# Autodesk Inventor assembly: ShooterAssembly_IFI-Flywheel
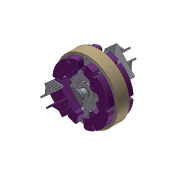
[picture p0: Inventor's stored thumbnail of the model, 180x180]
Saved by Autodesk Inventor 2012 (Build 160160000, 160)
## iProperties
Created: 2012-01-26
Part Number: ShooterAssembly_IFI-Flywheel
Document SubType Name: Assembly
Designer: JesseK
Mass: 2777.57 g
Surface Area: 4254.86 cm^2
Volume: 1099.46 cm^3
Density: 2.5263 g/cm^3
Author: JesseK
## Documents named in this file (6)
- Z:\UserData\Documents\Inventor\team1885frc\Robot2012\Shooter\ShooterAssembly_IFI-Flywheel.iam
- Z:\UserData\Documents\Inventor\team1885frc\Robot2012\Shooter\Axle_Shooter_8in.ipt
- Z:\UserData\Documents\Inventor\team1885frc\Robot2012\Shooter\IFI_FlyWheelAssembly_Jan23_Wide.iam
- Z:\UserData\Documents\Inventor\team1885frc\Hardware\Sprockets\Sprocket_Num25_25T_0.5bore.ipt
- Z:\UserData\Documents\Inventor\team1885frc\Robot2012\Shooter\BearingMount.ipt
- Z:\UserData\Documents\Inventor\team1885frc\Robot2012\Shooter\BearingMountBracket.ipt
## Components (9 placed, 5 different names)
1. Axle_Shooter_8in:1 — Mate:1, Flush:1, Mate:2, Mate:12, Mate:19, Flush:2, Flush:3
2. IFI_FlyWheelAssembly_Jan23_Wide:1 [sub-assembly] — Mate:1, Flush:1, Mate:5
3. Sprocket_Num25_25T_0.5bore:1 — Mate:2, Mate:5
4. BearingMount:1 — Mate:6, Mate:7, Mate:8, Mate:9, Mate:10, Mate:11, Mate:12, Flush:3, Mate:20
5. BearingMount:2 — Mate:13, Mate:14, Mate:15, Mate:16, Mate:17, Mate:18, Mate:19, Flush:2, Mate:20
6. BearingMountBracket:1 — Mate:6, Mate:10, Mate:11
7. BearingMountBracket:2 — Mate:7, Mate:8, Mate:9
8. BearingMountBracket:3 — Mate:14, Mate:15, Mate:16
9. BearingMountBracket:4 — Mate:13, Mate:17, Mate:18
## Relationships (21: Mate 18, Flush 3)
- Mate:1: Axle_Shooter_8in:1 ↔ IFI_FlyWheelAssembly_Jan23_Wide:1
- Flush:1 (31.75 mm): Axle_Shooter_8in:1 ↔ IFI_FlyWheelAssembly_Jan23_Wide:1
- Mate:2: Axle_Shooter_8in:1 ↔ Sprocket_Num25_25T_0.5bore:1
- Mate:5: IFI_FlyWheelAssembly_Jan23_Wide:1 ↔ Sprocket_Num25_25T_0.5bore:1
- Mate:6: BearingMount:1 ↔ BearingMountBracket:1
- Mate:7: BearingMount:1 ↔ BearingMountBracket:2
- Mate:8: BearingMount:1 ↔ BearingMountBracket:2
- Mate:9: BearingMount:1 ↔ BearingMountBracket:2
- Mate:10: BearingMount:1 ↔ BearingMountBracket:1
- Mate:11: BearingMount:1 ↔ BearingMountBracket:1
- Mate:12: Axle_Shooter_8in:1 ↔ BearingMount:1
- Mate:13: BearingMount:2 ↔ BearingMountBracket:4
- Mate:14: BearingMount:2 ↔ BearingMountBracket:3
- Mate:15: BearingMount:2 ↔ BearingMountBracket:3
- Mate:16: BearingMount:2 ↔ BearingMountBracket:3
- Mate:17: BearingMount:2 ↔ BearingMountBracket:4
- Mate:18: BearingMount:2 ↔ BearingMountBracket:4
- Mate:19: Axle_Shooter_8in:1 ↔ BearingMount:2
- Flush:2: Axle_Shooter_8in:1 ↔ BearingMount:2
- Flush:3: Axle_Shooter_8in:1 ↔ BearingMount:1
- Mate:20: BearingMount:1 ↔ BearingMount:2
